# Autodesk Inventor assembly: RescueKitThrow_Slope
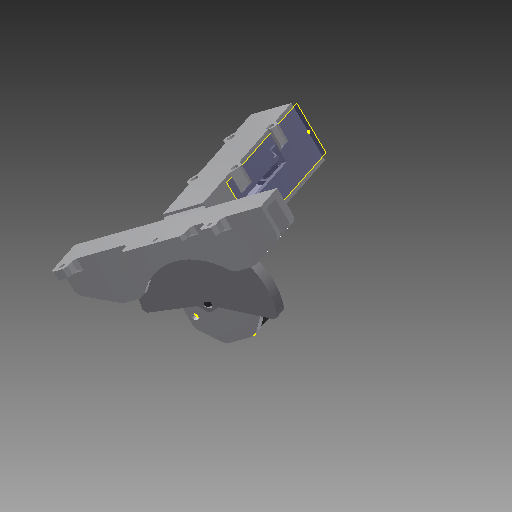
[picture p0: Inventor's stored thumbnail of the model, 512x512]
Saved by Autodesk Inventor 2018.3 (Build 223284000, 284)
## iProperties
Created: 2019-02-16
Part Number: RescueKitThrow_Slope
Material: 一般
Document SubType Name: Assembly
Designer: shun2
Author: shun2
## Documents named in this file (6)
- C:\Users\shun2\OneDrive\おそらく最新版(2018.7.31)\レスキューキット投下機構\RescueKitThrow_Slope.iam
- C:\Users\shun2\OneDrive\おそらく最新版(2018.7.31)\レスキューキット投下機構\RescueKitThrow_pipe.ipt
- C:\Users\shun2\OneDrive\おそらく最新版(2018.7.31)\レスキューキット投下機構\RescueKitThrow_slope.ipt
- C:\Users\shun2\OneDrive\おそらく最新版(2018.7.31)\レスキューキット投下機構\RescueKitThrow-Joint.ipt
- C:\Users\shun2\OneDrive\おそらく最新版(2018.7.31)\レスキューキット投下機構\RescueKitThrow_springholder.ipt
- C:\Users\shun2\OneDrive\おそらく最新版(2018.7.31)\レスキューキット投下機構\28BYJ-48.ipt
## Components (5 placed, 5 different names)
1. RescueKitThrow_pipe:1 — メイト:9, メイト:12, メイト:13, メイト:14, メイト:15
2. RescueKitThrow-Joint:1 — メイト:19, メイト:20
3. RescueKitThrow_slope:1 — メイト:9, メイト:12, メイト:13, メイト:14, メイト:16, メイト:17, メイト:18, メイト:20
4. RescueKitThrow_springholder:1 — メイト:15
5. 28BYJ-48:1 — メイト:16, メイト:17, メイト:18, メイト:19
## Relationships (10: Mate 10)
- メイト:9 [Mate]: RescueKitThrow_pipe:1 ↔ RescueKitThrow_slope:1
- メイト:12 [Mate]: RescueKitThrow_pipe:1 ↔ RescueKitThrow_slope:1
- メイト:13 [Mate] (0.5 mm): RescueKitThrow_pipe:1 ↔ RescueKitThrow_slope:1
- メイト:14 [Mate] (0.5 mm): RescueKitThrow_pipe:1 ↔ RescueKitThrow_slope:1
- メイト:15 [Mate]: RescueKitThrow_pipe:1 ↔ RescueKitThrow_springholder:1
- メイト:16 [Mate]: RescueKitThrow_slope:1 ↔ 28BYJ-48:1
- メイト:17 [Mate]: RescueKitThrow_slope:1 ↔ 28BYJ-48:1
- メイト:18 [Mate]: RescueKitThrow_slope:1 ↔ 28BYJ-48:1
- メイト:19 [Mate]: RescueKitThrow-Joint:1 ↔ 28BYJ-48:1
- メイト:20 [Mate] (0.5 mm): RescueKitThrow-Joint:1 ↔ RescueKitThrow_slope:1
